# Autodesk Inventor assembly: backplane
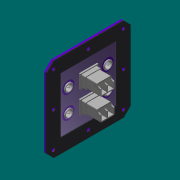
[picture p0: Inventor's stored thumbnail of the model, 180x180]
Saved by Autodesk Inventor 2016 SP1 (Build 200210100, 210)
## iProperties
Created: 2015-12-22
Part Number: backplane
Description: for SolidWorks
Document SubType Name: Assembly
Designer: sawai
Authority: Unknown
Sending System: Diptrace
Preprocessor: Open CASCADE STEP processor 6.6
Title: C:\Users\sawai\Desktop\backplane.step
Author: sawai
## Documents named in this file (7)
- C:\Users\sawai\OneDrive\projects\modularRICHBackplane\cad\backplane.iam
- C:\Users\sawai\OneDrive\projects\modularRICHBackplane\cad\backplane.ipt
- C:\Users\sawai\OneDrive\projects\modularRICHBackplane\cad\backplaneGasket.ipt
- C:\Users\sawai\OneDrive\projects\modularRICHBackplane\cad\connector\ERA.00.250.NTL\era_00_250_cll_01.ipt
- C:\Users\sawai\OneDrive\projects\modularRICHBackplane\cad\connector\ERA.00.250.NTL\era_00_250_cll_02.ipt
- C:\Users\sawai\OneDrive\projects\modularRICHBackplane\cad\connector\ERA.00.250.NTL\era_00_250_cll_03.ipt
- C:\Users\sawai\OneDrive\projects\modularRICHBackplane\cad\connector\lcLcCoupler.ipt
## Components (16 placed, 6 different names)
1. backplane:1 — Flush:1, Flush:2, Mate:2, Mate:3, Mate:6, Mate:7, Mate:8, Mate:9, Mate:10, Mate:11
2. backplaneGasket:1 — Flush:1, Flush:2, Mate:11
3. era_00_250_cll_03:1 — Mate:2, Mate:3, Mate:4, Mate:5
4. era_00_250_cll_01:1 — Mate:5, Mate:7
5. era_00_250_cll_02:1 — Mate:4, Mate:6
6. era_00_250_cll_03:2
7. era_00_250_cll_01:2
8. era_00_250_cll_02:2
9. era_00_250_cll_03:3
10. era_00_250_cll_01:3
11. era_00_250_cll_02:3
12. era_00_250_cll_03:4
13. era_00_250_cll_01:4
14. era_00_250_cll_02:4
15. lcLcCoupler:1 — Mate:8, Mate:9, Mate:10
16. lcLcCoupler:2
## Component patterns: (4 elements, first: era_00_250_cll_03:1 + era_00_250_cll_01:1 + era_00_250_cll_02:1), (2 elements, first: lcLcCoupler:1)
## Relationships (12: Mate 10, Flush 2)
- Flush:1: backplane:1 ↔ backplaneGasket:1
- Flush:2: backplane:1 ↔ backplaneGasket:1
- Mate:2: backplane:1 ↔ era_00_250_cll_03:1
- Mate:3: backplane:1 ↔ era_00_250_cll_03:1
- Mate:4: era_00_250_cll_03:1 ↔ era_00_250_cll_02:1
- Mate:5: era_00_250_cll_03:1 ↔ era_00_250_cll_01:1
- Mate:6: backplane:1 ↔ era_00_250_cll_02:1
- Mate:7 (1 mm): backplane:1 ↔ era_00_250_cll_01:1
- Mate:8 (0.125 mm): backplane:1 ↔ lcLcCoupler:1
- Mate:9 (0.125 mm): backplane:1 ↔ lcLcCoupler:1
- Mate:10: backplane:1 ↔ lcLcCoupler:1
- Mate:11: backplane:1 ↔ backplaneGasket:1
